# Autodesk Inventor assembly: W520
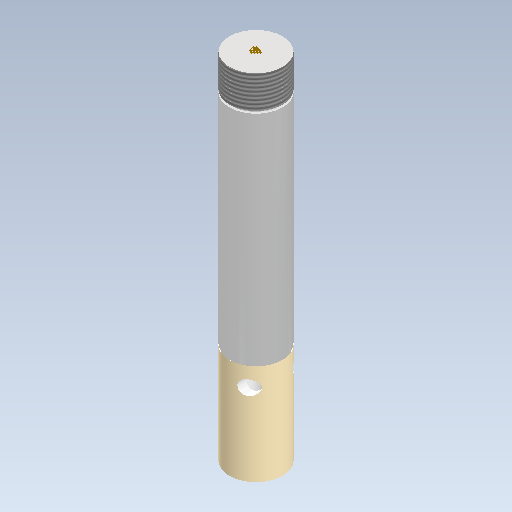
[picture p0: Inventor's stored thumbnail of the model, 512x512]
Saved by Autodesk Inventor 2020 (Build 240168000, 168)
## iProperties
Created: 2021-10-16
Part Number: W520
Document SubType Name: Assembly
Designer: DANIEL
Author: DANIEL
## Documents named in this file (3)
- C:\Users\DANIEL\Documents\Personal\Convocatorias\Escollera\tesis\CAD\W520.iam
- C:\Users\DANIEL\Documents\Personal\Convocatorias\Escollera\tesis\CAD\W520inferior.ipt
- C:\Users\DANIEL\Documents\Personal\Convocatorias\Escollera\tesis\CAD\W520superior.ipt
## Components (2 placed, 2 different names)
1. W520inferior:1 — Rígido:1
2. W520superior:1 — Rígido:1
## Relationships (1: WeldJoint 1)
- Rígido:1 [WeldJoint]: W520inferior:1 ↔ W520superior:1
